# Autodesk Inventor assembly: nhk37
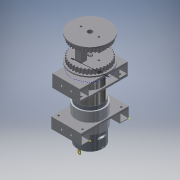
[picture p0: Inventor's stored thumbnail of the model, 180x180]
Saved by Autodesk Inventor 2019 (Build 230136000, 136)
## iProperties
Created: 2022-02-27
Part Number: nhk37
Material: 一般
Document SubType Name: Assembly
Designer: yuta
Author: yuta
## Documents named in this file (3)
- C:\Users\yuta\Documents\NHK\nhk37.iam
- C:\Users\yuta\Documents\NHK\nhk35.iam
- C:\Users\yuta\Documents\NHK\nhk36.iam
## Components (2 placed, 2 different names)
1. nhk35:1 [sub-assembly] — メイト:1, メイト:2, メイト:3
2. nhk36:1 [sub-assembly] — メイト:1, メイト:2, メイト:3
## Relationships (3: Mate 3)
- メイト:1 [Mate]: nhk35:1 ↔ nhk36:1
- メイト:2 [Mate]: nhk35:1 ↔ nhk36:1
- メイト:3 [Mate]: nhk35:1 ↔ nhk36:1
